# Autodesk Inventor assembly: Hatch design
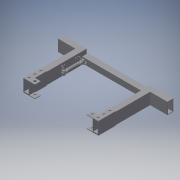
[picture p0: Inventor's stored thumbnail of the model, 180x180]
Saved by Autodesk Inventor 2018 (Build 220112000, 112)
## iProperties
Created: 2019-01-16
Part Number: Hatch design
Document SubType Name: Assembly
Designer: s-4008082
Author: s-4008082
## Documents named in this file (6)
- C:\Users\Burni\Desktop\Robotics\hatch\Hatch design.iam
- C:\Users\Burni\Desktop\Robotics\hatch\left arm.ipt
- C:\Users\Burni\Desktop\Robotics\hatch\right arm.ipt
- C:\Users\Burni\Desktop\Robotics\hatch\push bar.ipt
- C:\Users\Burni\Desktop\Robotics\hatch\PARTserver02019011803125824465437192d056f\AIS2018\021-DXP(F,D-770).iam
- C:\Users\Burni\Desktop\Robotics\hatch\bracing 2x3.ipt
## Components (9 placed, 5 different names)
1. left arm:1 — Mate:15, Mate:16, Flush:8, Flush:9, Flush:11, Mate:22, Mate:23, Flush:12, Flush:13, Mate:24, Flush:14, Flush:15
2. right arm:1 — Mate:17, Flush:10, Mate:18, Mate:19, Mate:20, Mate:21
3. push bar:1 — Mate:15
4. 021-DXP(F,D-770):1 [sub-assembly] — Mate:16, Flush:8, Flush:9
5. 021-DXP(F,D-770):2 [sub-assembly] — Mate:17, Flush:10
6. bracing 2x3:1 — Flush:11, Mate:22, Mate:23
7. bracing 2x3:2 — Flush:12, Flush:13, Mate:24, Flush:14, Flush:15
8. bracing 2x3:3 — Mate:20, Mate:21
9. bracing 2x3:4 — Mate:18, Mate:19
## Relationships (18: Mate 10, Flush 8)
- Mate:15 (6.35 mm): left arm:1 ↔ push bar:1
- Mate:16: left arm:1 ↔ 021-DXP(F,D-770):1
- Flush:8 (34.925 mm): left arm:1 ↔ 021-DXP(F,D-770):1
- Flush:9 (11.43 mm): left arm:1 ↔ 021-DXP(F,D-770):1
- Mate:17: right arm:1 ↔ 021-DXP(F,D-770):2
- Flush:10 (34.925 mm): right arm:1 ↔ 021-DXP(F,D-770):2
- Mate:18: right arm:1 ↔ bracing 2x3:4
- Mate:19: right arm:1 ↔ bracing 2x3:4
- Mate:20: right arm:1 ↔ bracing 2x3:3
- Mate:21: right arm:1 ↔ bracing 2x3:3
- Flush:11: left arm:1 ↔ bracing 2x3:1
- Mate:22: left arm:1 ↔ bracing 2x3:1
- Mate:23: left arm:1 ↔ bracing 2x3:1
- Flush:12: left arm:1 ↔ bracing 2x3:2
- Flush:13: left arm:1 ↔ bracing 2x3:2
- Mate:24: left arm:1 ↔ bracing 2x3:2
- Flush:14: left arm:1 ↔ bracing 2x3:2
- Flush:15: left arm:1 ↔ bracing 2x3:2
